# Autodesk Inventor assembly: Assembly2
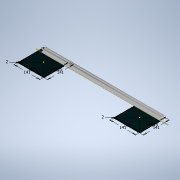
[picture p0: Inventor's stored thumbnail of the model, 180x180]
Saved by Autodesk Inventor 2021 (Build 250183000, 183)
## iProperties
Created: 2023-12-15
Part Number: Assembly2
Document SubType Name: Assembly
Designer: assman
Author: assman
## Documents named in this file (4)
- C:\dev\3DModels\3party\daisq\Assembly2.iam
- C:\dev\3DModels\3party\daisq\Part1.ipt
- C:\dev\3DModels\3party\alu_profiles\misc\20x20 aluminum.ipt
- C:\dev\3DModels\3party\daisq\plate_f16.ipt
## Components (4 placed, 3 different names)
1. Part1:1
2. 20x20 aluminum:1 — Mate:1, Mate:2
3. plate_f16:1 — Mate:1
4. plate_f16:2 — Mate:2
## Relationships (2: Mate 2)
- Mate:1: 20x20 aluminum:1 ↔ plate_f16:1
- Mate:2: 20x20 aluminum:1 ↔ plate_f16:2
